# Autodesk Inventor assembly: Zespół1
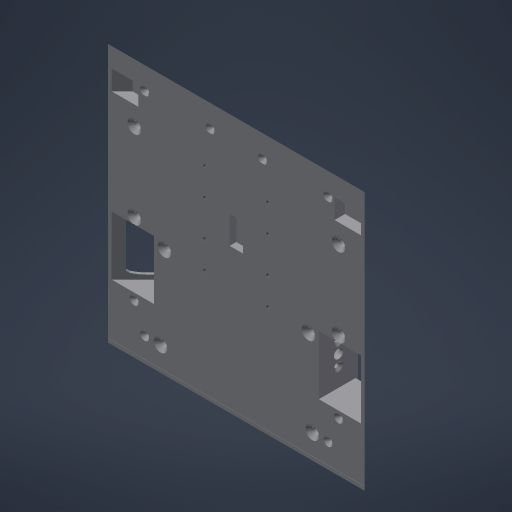
[picture p0: Inventor's stored thumbnail of the model, 512x512]
Saved by Autodesk Inventor 2023 (Build 270158000, 158)
## iProperties
Created: 2021-11-14
Part Number: Zespół1
Material: Ogólny
Document SubType Name: Assembly
Designer: Michał
Author: Michał
## Documents named in this file (14)
- D:\Projekty\RoboIlo\Piramida\3D\Zespół1.iam
- D:\Projekty\RoboIlo\Piramida\3D\blacha.ipt
- D:\Projekty\RoboIlo\Piramida\3D\mocowanie_silnika_wariant1.ipt
- D:\Projekty\RoboIlo\Piramida\3D\MocowanieCzujnikaBezScianki.ipt
- D:\Projekty\RoboIlo\Piramida\3D\MocowanieBok2.ipt
- D:\Projekty\RoboIlo\Piramida\3D\mocowanie_silnika_wariant1_MIR.ipt
- D:\Projekty\RoboIlo\Piramida\3D\MocowanieBok2_MIR.ipt
- D:\Projekty\RoboIlo\Piramida\3D\MocowanieCzujnikaBazSciankiLewy.ipt
- D:\Projekty\RoboIlo\Piramida\3D\Bok2mm.ipt
- D:\Projekty\RoboIlo\Piramida\3D\Przod2mm.ipt
- D:\Projekty\RoboIlo\Piramida\3D\Bok2mm_MIR.ipt
- D:\Projekty\RoboIlo\Piramida\3D\Tyl.ipt
- D:\Projekty\RoboIlo\Piramida\3D\PlogPiramida.ipt
- D:\Projekty\RoboIlo\Piramida\3D\Dach.ipt
## Components (13 placed, 13 different names)
1. blacha:1 — Wstaw:1, Wstaw:2, Wstaw:6, Zestawiający:1, Zestawiający:2, Zestawiający:3, Wstaw:19, Wstaw:20, Wstaw:27, Wstaw:28, Wstaw:29, Wstaw:30, Wstaw:41, Wstaw:42
2. MocowanieCzujnikaBezScianki:1 — Wstaw:1, Wstaw:2, Wstaw:5, Wstaw:37, Wstaw:38
3. mocowanie_silnika_wariant1:1 — Wstaw:5, Wstaw:6, Wstaw:35
4. MocowanieBok2:1 — Wstaw:27, Wstaw:28
5. mocowanie_silnika_wariant1_MIR:1 — Wstaw:19, Wstaw:21, Wstaw:36, Równoległy:1
6. MocowanieBok2_MIR:1 — Wstaw:29, Wstaw:30
7. MocowanieCzujnikaBazSciankiLewy:1 — Wstaw:20, Wstaw:21, Wstaw:33, Wstaw:34
8. Bok2mm:1 — Wstaw:33, Wstaw:34
9. Bok2mm_MIR:1 — Wstaw:37, Wstaw:38
10. Tyl:1 — Wstaw:35, Wstaw:36
11. PlogPiramida:1 — Wstaw:41, Wstaw:42
12. Przod2mm:1
13. Dach:1 — Równoległy:1
## Relationships (23: Insert 19, Mate 3, Flush 1)
- Wstaw:1 [Insert]: blacha:1 ↔ MocowanieCzujnikaBezScianki:1
- Wstaw:2 [Insert]: blacha:1 ↔ MocowanieCzujnikaBezScianki:1
- Wstaw:5 [Insert]: MocowanieCzujnikaBezScianki:1 ↔ mocowanie_silnika_wariant1:1
- Wstaw:6 [Insert]: blacha:1 ↔ mocowanie_silnika_wariant1:1
- Zestawiający:1 [Mate]: blacha:1
- Zestawiający:2 [Mate]: blacha:1
- Zestawiający:3 [Mate]: blacha:1
- Wstaw:19 [Insert]: blacha:1 ↔ mocowanie_silnika_wariant1_MIR:1
- Wstaw:20 [Insert]: blacha:1 ↔ MocowanieCzujnikaBazSciankiLewy:1
- Wstaw:21 [Insert]: mocowanie_silnika_wariant1_MIR:1 ↔ MocowanieCzujnikaBazSciankiLewy:1
- Wstaw:27 [Insert]: blacha:1 ↔ MocowanieBok2:1
- Wstaw:28 [Insert]: blacha:1 ↔ MocowanieBok2:1
- Wstaw:29 [Insert]: blacha:1 ↔ MocowanieBok2_MIR:1
- Wstaw:30 [Insert]: blacha:1 ↔ MocowanieBok2_MIR:1
- Wstaw:33 [Insert]: MocowanieCzujnikaBazSciankiLewy:1 ↔ Bok2mm:1
- Wstaw:34 [Insert]: MocowanieCzujnikaBazSciankiLewy:1 ↔ Bok2mm:1
- Wstaw:35 [Insert]: mocowanie_silnika_wariant1:1 ↔ Tyl:1
- Wstaw:36 [Insert]: mocowanie_silnika_wariant1_MIR:1 ↔ Tyl:1
- Wstaw:37 [Insert]: MocowanieCzujnikaBezScianki:1 ↔ Bok2mm_MIR:1
- Wstaw:38 [Insert]: MocowanieCzujnikaBezScianki:1 ↔ Bok2mm_MIR:1
- Wstaw:41 [Insert]: blacha:1 ↔ PlogPiramida:1
- Wstaw:42 [Insert]: blacha:1 ↔ PlogPiramida:1
- Równoległy:1 [Flush]: mocowanie_silnika_wariant1_MIR:1 ↔ Dach:1
